# Autodesk Inventor assembly: Z_PLATE
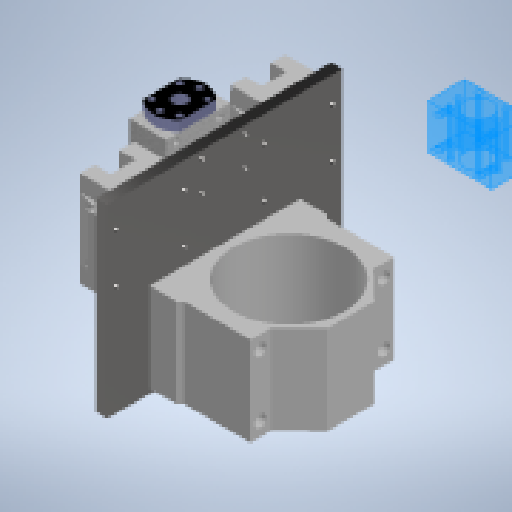
[picture p0: Inventor's stored thumbnail of the model, 512x512]
Saved by Autodesk Inventor 2023 (Build 270158000, 158)
## iProperties
Created: 2022-05-07
Part Number: Z_PLATE
Document SubType Name: Assembly
Designer: plebbb
Author: plebbb
## Documents named in this file (4)
- D:\Users\plebbb\Desktop\CNC_Project\Z_PLATE.iam
- D:\Users\plebbb\Desktop\CNC_Project\HGW20CC_Slider.ipt
- D:\Users\plebbb\Desktop\CNC_Project\Spindle_Mounting_Plate.ipt
- D:\Users\plebbb\Desktop\CNC_Project\Spindle_Holder.ipt
## Components (4 placed, 3 different names)
1. HGW20CC_Slider:1 — Angle:1
2. HGW20CC_Slider:2 — Mate:14, Angle:2
3. Spindle_Mounting_Plate:1 — Angle:1, Mate:14, Angle:2
4. Spindle_Holder:1
## Relationships (9: Mate 7, Angle 2)
- [Mate]: HGW20CC_Slider:2 ↔ Spindle_Mounting_Plate:1
- [Mate]: HGW20CC_Slider:1 ↔ Spindle_Mounting_Plate:1
- [Mate]: HGW20CC_Slider:1 ↔ Spindle_Mounting_Plate:1
- [Mate]: Spindle_Mounting_Plate:1 ↔ Spindle_Holder:1
- [Mate]: Spindle_Mounting_Plate:1 ↔ Spindle_Holder:1
- [Mate]: Spindle_Mounting_Plate:1 ↔ Spindle_Holder:1
- Angle:1 (180 deg): HGW20CC_Slider:1 ↔ Spindle_Mounting_Plate:1
- Mate:14: HGW20CC_Slider:2 ↔ Spindle_Mounting_Plate:1
- Angle:2 (180 deg): HGW20CC_Slider:2 ↔ Spindle_Mounting_Plate:1
